# Autodesk Inventor assembly: AssamblyRobot
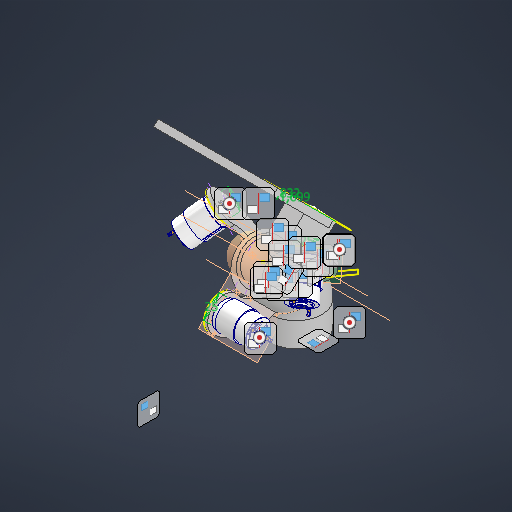
[picture p0: Inventor's stored thumbnail of the model, 512x512]
Saved by Autodesk Inventor 2026 (Build 300175050, 175E)
## iProperties
Created: 2025-07-17
Part Number: AssamblyRobot
Document SubType Name: Assembly
Designer: RubenPC
Author: RubenPC
## Documents named in this file (6)
- C:\Users\RubenPC\Code\RoboTT\AssamblyRobot.iam
- C:\Users\RubenPC\Code\RoboTT\assets\MABUCHI_MOTOR_385\MABUCHI_MOTOR_385\MABUCHI_MOTOR_385.ipt
- C:\Users\RubenPC\Code\RoboTT\assets\4880K691_Standard-Wall PVC Pipe Fitting for Water\4880K691_Standard-Wall PVC Pipe Fitting for Water\4880K691_Standard-Wall PVC Pipe Fitting for Water.ipt
- C:\Users\RubenPC\OneDrive\Documentos\Wheel.ipt
- C:\Users\RubenPC\Code\RoboTT\Ball.ipt
- C:\Users\RubenPC\Code\RoboTT\Head3MotorsSustain.ipt
## Components (9 placed, 5 different names)
1. MABUCHI_MOTOR_385:1 — Mate:3, Mate:8, Mate:10, Flush:5
2. MABUCHI_MOTOR_385:2 — Mate:5, Mate:6
3. MABUCHI_MOTOR_385:3 — Mate:2, Mate:7, Mate:11, Flush:6
4. 4880K691_Standard-Wall PVC Pipe Fitting for Water:1 — Mate:1, Mate:2, Mate:3, Flush:1, Flush:2, Mate:5, Mate:6, Mate:7, Mate:8, Mate:9, Mate:12, Mate:13, Mate:14, Mate:15, Mate:16, Mate:17, Mate:18, Flush:8, Mate:20
5. Wheel:1 — Flush:3, Flush:4
6. Wheel:2 — Mate:11
7. Wheel:3 — Mate:10
8. Ball:1 — Mate:18
9. Head3MotorsSustain:1 — Flush:5, Flush:6, Flush:8, Mate:20
## Relationships (26: Mate 19, Flush 7)
- Mate:1: 4880K691_Standard-Wall PVC Pipe Fitting for Water:1
- Mate:2: MABUCHI_MOTOR_385:3 ↔ 4880K691_Standard-Wall PVC Pipe Fitting for Water:1
- Mate:3: MABUCHI_MOTOR_385:1 ↔ 4880K691_Standard-Wall PVC Pipe Fitting for Water:1
- Flush:1: 4880K691_Standard-Wall PVC Pipe Fitting for Water:1
- Mate:4
- Flush:2: 4880K691_Standard-Wall PVC Pipe Fitting for Water:1
- Mate:5: MABUCHI_MOTOR_385:2 ↔ 4880K691_Standard-Wall PVC Pipe Fitting for Water:1
- Mate:6: MABUCHI_MOTOR_385:2 ↔ 4880K691_Standard-Wall PVC Pipe Fitting for Water:1
- Mate:7: MABUCHI_MOTOR_385:3 ↔ 4880K691_Standard-Wall PVC Pipe Fitting for Water:1
- Mate:8: MABUCHI_MOTOR_385:1 ↔ 4880K691_Standard-Wall PVC Pipe Fitting for Water:1
- Mate:9: 4880K691_Standard-Wall PVC Pipe Fitting for Water:1
- Flush:3: Wheel:1
- Flush:4: Wheel:1
- Mate:10: MABUCHI_MOTOR_385:1 ↔ Wheel:3
- Mate:11: MABUCHI_MOTOR_385:3 ↔ Wheel:2
- Mate:12: 4880K691_Standard-Wall PVC Pipe Fitting for Water:1
- Mate:13: 4880K691_Standard-Wall PVC Pipe Fitting for Water:1
- Mate:14: 4880K691_Standard-Wall PVC Pipe Fitting for Water:1
- Mate:15: 4880K691_Standard-Wall PVC Pipe Fitting for Water:1
- Mate:16: 4880K691_Standard-Wall PVC Pipe Fitting for Water:1
- Mate:17: 4880K691_Standard-Wall PVC Pipe Fitting for Water:1
- Mate:18: 4880K691_Standard-Wall PVC Pipe Fitting for Water:1 ↔ Ball:1
- Flush:5: MABUCHI_MOTOR_385:1 ↔ Head3MotorsSustain:1
- Flush:6: MABUCHI_MOTOR_385:3 ↔ Head3MotorsSustain:1
- Flush:8: 4880K691_Standard-Wall PVC Pipe Fitting for Water:1 ↔ Head3MotorsSustain:1
- Mate:20: 4880K691_Standard-Wall PVC Pipe Fitting for Water:1 ↔ Head3MotorsSustain:1
